# Autodesk Inventor assembly: PVC_Catapult
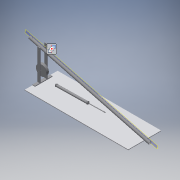
[picture p0: Inventor's stored thumbnail of the model, 180x180]
Saved by Autodesk Inventor 2016 SP1 (Build 200210100, 210)
## iProperties
Created: 2016-01-12
Part Number: PVC_Catapult
Document SubType Name: Assembly
Designer: steele
Author: steele
## Documents named in this file (8)
- C:\snobotics\CAD-Development\robSteele\SnoBotics2016\FirstCutCatapult\PVC_Catapult.iam
- C:\snobotics\CAD-Development\robSteele\SnoBotics2016\FirstCutCatapult\CatapultBase.ipt
- C:\snobotics\CAD-Development\robSteele\SnoBotics2016\FirstCutCatapult\cPvcSupport.ipt
- C:\snobotics\CAD-Development\robSteele\SnoBotics2016\FirstCutCatapult\catapultMaxVolume.ipt
- C:\snobotics\CAD-Development\robSteele\SnoBotics2016\FirstCutCatapult\CatapultAxel.ipt
- C:\snobotics\CAD-Development\robSteele\SnoBotics2016\FirstCutCatapult\roundCatapultArm.ipt
- C:\snobotics\CAD-MfgResources\McMaster-Carr\Air Cylinder\Universal Mount\Single Acting Spring Return\3_4 bore 6 stroke\6498K045.ipt
- C:\snobotics\CAD-Development\robSteele\SnoBotics2016\FirstCutCatapult\cArmPully.ipt
## Components (10 placed, 7 different names)
1. CatapultBase:1 — Mate:1, Flush:1, Mate:2, Mate:3, Flush:2, Mate:4, Mate:5, Flush:3
2. cPvcSupport:1 — Mate:1, Flush:1, Mate:2, Insert:1, Insert:2
3. cPvcSupport:2 — Mate:3, Flush:2, Mate:4
4. catapultMaxVolume:1 — Mate:5, Flush:3, Mate:6
5. CatapultAxel:1 — Insert:1, Mate:7, Mate:11
6. roundCatapultArm:1 — Mate:7, Mate:8
7. CatapultAxel:2 — Insert:2, Mate:9
8. 6498K045:1
9. cArmPully:1 — Mate:9, Mate:10
10. roundCatapultArm:2 — Mate:11, Mate:12
## Relationships (17: Mate 12, Flush 3, Insert 2)
- Mate:1: CatapultBase:1 ↔ cPvcSupport:1
- Flush:1 (76.2 mm): CatapultBase:1 ↔ cPvcSupport:1
- Mate:2: CatapultBase:1 ↔ cPvcSupport:1
- Mate:3: CatapultBase:1 ↔ cPvcSupport:2
- Flush:2 (76.2 mm): CatapultBase:1 ↔ cPvcSupport:2
- Mate:4: CatapultBase:1 ↔ cPvcSupport:2
- Mate:5: CatapultBase:1 ↔ catapultMaxVolume:1
- Flush:3: CatapultBase:1 ↔ catapultMaxVolume:1
- Mate:6: catapultMaxVolume:1
- Insert:1: cPvcSupport:1 ↔ CatapultAxel:1
- Mate:7: CatapultAxel:1 ↔ roundCatapultArm:1
- Mate:8: roundCatapultArm:1
- Insert:2: cPvcSupport:1 ↔ CatapultAxel:2
- Mate:9: CatapultAxel:2 ↔ cArmPully:1
- Mate:10: cArmPully:1
- Mate:11: CatapultAxel:1 ↔ roundCatapultArm:2
- Mate:12: roundCatapultArm:2
